# Autodesk Inventor assembly: HB_armMountU03
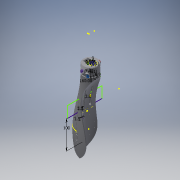
[picture p0: Inventor's stored thumbnail of the model, 180x180]
Saved by Autodesk Inventor 2016 (Build 200138000, 138)
## iProperties
Created: 2015-02-09
Part Number: HB_armMountU03
Document SubType Name: Assembly
Designer: Yamaura
Author: Yamaura
## Documents named in this file (17)
- C:\Users\Yamaura\Documents\GitHub\HACKberry\HACKberry-hardware\3D\Inventor\Parts\HB_armMountU03.iam
- C:\Users\Yamaura\Documents\GitHub\HACKberry\HACKberry-hardware\3D\Inventor\Parts\SBI-SUJ-1d4.ipt
- C:\Users\Yamaura\Documents\GitHub\HACKberry\HACKberry-hardware\3D\Inventor\Parts\CP 0.5-6-8.ipt
- C:\Users\Yamaura\Documents\GitHub\HACKberry\HACKberry-hardware\3D\Inventor\Parts\HBpronationLockPin02.ipt
- C:\Users\Yamaura\Documents\GitHub\HACKberry\HACKberry-hardware\3D\Inventor\Parts\HBlockPlateHolder02.ipt
- C:\Users\Yamaura\Documents\GitHub\HACKberry\HACKberry-hardware\3D\Inventor\Parts\HBabductionLever02.ipt
- C:\Users\Yamaura\Documents\GitHub\HACKberry\HACKberry-hardware\3D\Inventor\Parts\HBejectorLever02.ipt
- C:\Users\Yamaura\Documents\GitHub\HACKberry\HACKberry-hardware\3D\Inventor\Parts\HBarmMount02.ipt
- C:\Users\Yamaura\Google ドライブ\exiii\3D\150405HackBerry\00_Latest\HbMainFrame03.ipt
- C:\Users\Yamaura\Documents\GitHub\HACKberry\HACKberry-hardware\3D\Inventor\Parts\150404Morikawa.ipt
- C:\Users\Yamaura\Documents\GitHub\HACKberry\HACKberry-hardware\3D\Inventor\Parts\ScrewM3L8Btite.ipt
- C:\Users\Yamaura\Documents\GitHub\HACKberry\HACKberry-hardware\3D\Inventor\Parts\HBarmMountBaseCover03.ipt
- C:\Users\Yamaura\Documents\GitHub\HACKberry\HACKberry-hardware\3D\Inventor\Parts\HBarmMountBase03.ipt
- C:\Users\Yamaura\Documents\GitHub\HACKberry\HACKberry-hardware\3D\Inventor\Parts\HbSocketU02.iam
- C:\Users\Yamaura\Documents\GitHub\HACKberry\HACKberry-hardware\3D\Inventor\Parts\HbSocketU03.iam
- C:\Users\Yamaura\Documents\GitHub\HACKberry\HACKberry-hardware\3D\Inventor\Parts\flatScrewM2L6PHI3.3T1.3.ipt
- C:\Users\Yamaura\Documents\GitHub\HACKberry\HACKberry-hardware\3D\Inventor\Parts\ScrewM2L10.ipt
## Components (32 placed, 16 different names)
1. flatScrewM2L6PHI3.3T1.3:1
2. flatScrewM2L6PHI3.3T1.3:2
3. SBI-SUJ-1d4:1
4. CP 0.5-6-8:1 — メイト:56, メイト:57
5. CP 0.5-6-8:2
6. CP 0.5-6-8:3
7. CP 0.5-6-8:4
8. HBpronationLockPin02:1
9. HBlockPlateHolder02:1 — メイト:4, メイト:5, メイト:6, メイト:78, メイト:79
10. HBarmMountBaseCover03:1 — メイト:74, メイト:75, 角度:4
11. HbMainFrame03:1 — メイト:3, メイト:4, メイト:5, メイト:6, 角度:1
12. HBabductionLever02:1 — 角度:2, メイト:56, メイト:80
13. HBejectorLever02:1 — メイト:57, メイト:81, メイト:82
14. HBarmMount02:1 — メイト:81, メイト:82
15. 150404Morikawa:1
16. ScrewM3L8Btite:1
17. ScrewM3L8Btite:2
18. HBarmMountBase03:1 — メイト:76, フラッシュ:14, メイト:77, メイト:80
19. HbSocketU02:1 [sub-assembly] — フラッシュ:15, フラッシュ:16, フラッシュ:17, メイト:83, メイト:84, メイト:85, メイト:86, メイト:87, メイト:88, メイト:89, メイト:90, メイト:91, メイト:92, メイト:93, メイト:94, フラッシュ:18, メイト:95, メイト:96, メイト:97, メイト:98, メイト:99, メイト:100, フラッシュ:19, フラッシュ:20, フラッシュ:21, フラッシュ:22, フラッシュ:23
20. HbSocketU03:1 [sub-assembly] — メイト:77, メイト:78, メイト:79
21. ScrewM2L10:1 — メイト:83, メイト:84
22. ScrewM2L10:2 — メイト:85, メイト:86
23. ScrewM2L10:3 — メイト:87, メイト:88
24. ScrewM2L10:4 — メイト:89, メイト:90
25. ScrewM2L10:5 — メイト:91, メイト:92
26. ScrewM2L10:6 — メイト:93, メイト:94
27. flatScrewM2L6PHI3.3T1.3:3 — フラッシュ:18, メイト:95
28. flatScrewM2L6PHI3.3T1.3:4 — メイト:99, フラッシュ:22
29. flatScrewM2L6PHI3.3T1.3:5 — メイト:100, フラッシュ:23
30. flatScrewM2L6PHI3.3T1.3:6 — メイト:98, フラッシュ:21
31. flatScrewM2L6PHI3.3T1.3:7 — メイト:97, フラッシュ:20
32. flatScrewM2L6PHI3.3T1.3:8 — メイト:96, フラッシュ:19
## Relationships (46: Mate 33, Flush 10, Angle 3)
- メイト:3 [Mate]: HbMainFrame03:1
- メイト:4 [Mate]: HBlockPlateHolder02:1 ↔ HbMainFrame03:1
- メイト:5 [Mate]: HBlockPlateHolder02:1 ↔ HbMainFrame03:1
- メイト:6 [Mate]: HBlockPlateHolder02:1 ↔ HbMainFrame03:1
- 角度:1 [Angle] (90 deg): HbMainFrame03:1
- 角度:2 [Angle] (0 deg): HBabductionLever02:1
- メイト:56 [Mate]: CP 0.5-6-8:1 ↔ HBabductionLever02:1
- メイト:57 [Mate]: CP 0.5-6-8:1 ↔ HBejectorLever02:1
- メイト:74 [Mate]: HBarmMountBaseCover03:1
- メイト:75 [Mate] (9.2 mm): HBarmMountBaseCover03:1
- 角度:4 [Angle] (0 deg): HBarmMountBaseCover03:1
- メイト:76 [Mate]: HBarmMountBase03:1
- フラッシュ:14 [Flush] (-9.2 mm): HBarmMountBase03:1
- フラッシュ:15 [Flush]: HbSocketU02:1
- フラッシュ:16 [Flush]: HbSocketU02:1
- フラッシュ:17 [Flush]: HbSocketU02:1
- メイト:77 [Mate]: HBarmMountBase03:1 ↔ HbSocketU03:1
- メイト:78 [Mate]: HBlockPlateHolder02:1 ↔ HbSocketU03:1
- メイト:79 [Mate]: HBlockPlateHolder02:1 ↔ HbSocketU03:1
- メイト:80 [Mate] (0.5 mm): HBabductionLever02:1 ↔ HBarmMountBase03:1
- メイト:81 [Mate] (0.5 mm): HBejectorLever02:1 ↔ HBarmMount02:1
- メイト:82 [Mate]: HBejectorLever02:1 ↔ HBarmMount02:1
- メイト:83 [Mate]: HbSocketU02:1 ↔ ScrewM2L10:1
- メイト:84 [Mate]: HbSocketU02:1 ↔ ScrewM2L10:1
- メイト:85 [Mate]: HbSocketU02:1 ↔ ScrewM2L10:2
- メイト:86 [Mate]: HbSocketU02:1 ↔ ScrewM2L10:2
- メイト:87 [Mate]: HbSocketU02:1 ↔ ScrewM2L10:3
- メイト:88 [Mate]: HbSocketU02:1 ↔ ScrewM2L10:3
- メイト:89 [Mate]: HbSocketU02:1 ↔ ScrewM2L10:4
- メイト:90 [Mate]: HbSocketU02:1 ↔ ScrewM2L10:4
- メイト:91 [Mate]: HbSocketU02:1 ↔ ScrewM2L10:5
- メイト:92 [Mate]: HbSocketU02:1 ↔ ScrewM2L10:5
- メイト:93 [Mate]: HbSocketU02:1 ↔ ScrewM2L10:6
- メイト:94 [Mate]: HbSocketU02:1 ↔ ScrewM2L10:6
- フラッシュ:18 [Flush] (-1.2 mm): HbSocketU02:1 ↔ flatScrewM2L6PHI3.3T1.3:3
- メイト:95 [Mate]: HbSocketU02:1 ↔ flatScrewM2L6PHI3.3T1.3:3
- メイト:96 [Mate]: HbSocketU02:1 ↔ flatScrewM2L6PHI3.3T1.3:8
- メイト:97 [Mate]: HbSocketU02:1 ↔ flatScrewM2L6PHI3.3T1.3:7
- メイト:98 [Mate]: HbSocketU02:1 ↔ flatScrewM2L6PHI3.3T1.3:6
- メイト:99 [Mate]: HbSocketU02:1 ↔ flatScrewM2L6PHI3.3T1.3:4
- メイト:100 [Mate]: HbSocketU02:1 ↔ flatScrewM2L6PHI3.3T1.3:5
- フラッシュ:19 [Flush] (1.2 mm): HbSocketU02:1 ↔ flatScrewM2L6PHI3.3T1.3:8
- フラッシュ:20 [Flush] (-1.2 mm): HbSocketU02:1 ↔ flatScrewM2L6PHI3.3T1.3:7
- フラッシュ:21 [Flush] (-1.2 mm): HbSocketU02:1 ↔ flatScrewM2L6PHI3.3T1.3:6
- フラッシュ:22 [Flush] (-1.2 mm): HbSocketU02:1 ↔ flatScrewM2L6PHI3.3T1.3:4
- フラッシュ:23 [Flush] (-1.2 mm): HbSocketU02:1 ↔ flatScrewM2L6PHI3.3T1.3:5
